# Autodesk Inventor assembly: 810003-XX
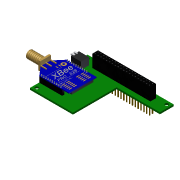
[picture p0: Inventor's stored thumbnail of the model, 180x180]
Saved by Autodesk Inventor 2015 (Build 190159000, 159)
## iProperties
Created: 2014-08-12
Part Number: 810003-XX
Document SubType Name: Assembly
Designer: david
Author: david
## Documents named in this file (6)
- C:\SharedDrive\Dropbox\FAST Robotics\Products\810003_Radio Shield\MECH\810003_Radio Shield\810003A\810003-XX.iam
- C:\SharedDrive\Dropbox\FAST Robotics\Products\810003_Radio Shield\MECH\818001_Radio Shield Bare PCB\818001A\818001A_Radio Shield Bare PCB.ipt
- C:\SharedDrive\Dropbox\FAST Robotics\Library\784005_HEADER Female Socket 10pos 2mm Thru-Hole\784005_HEADER Female Socket 10pos 2mm Thru-Hole.ipt
- C:\SharedDrive\Dropbox\FAST Robotics\Library\616001_DIP Switch Side 2Pos\MECH\616001_DIP Switch Side 2Pos.ipt
- C:\SharedDrive\Dropbox\FAST Robotics\Library\363002_XBee XBP24BZ7SIT\MECH\Imported Components\User Library-XBP24BZ7SIT-004-radio\Assembly2.iam
- C:\SharedDrive\Dropbox\FAST Robotics\Library\784009_PC104 Connector\784009_PC104 Connector.ipt
## Components (6 placed, 5 different names)
1. 818001A_Radio Shield Bare PCB:1 — Flush:1, Flush:2, Flush:3, Mate:3, Mate:4, Flush:14, Flush:15, Flush:16, Flush:17, Mate:9, Flush:18, Mate:10
2. 784005_HEADER Female Socket 10pos 2mm Thru-Hole:1 — Flush:10, Mate:3, Mate:5, Mate:6, Flush:13, Flush:14, Flush:15, Mate:8
3. 784005_HEADER Female Socket 10pos 2mm Thru-Hole:2 — Flush:10, Flush:13, Mate:7
4. 616001_DIP Switch Side 2Pos:1 — Mate:4, Flush:16, Flush:17
5. Assembly2:1 [sub-assembly] — Mate:5, Mate:6, Mate:7, Mate:8
6. 784009_PC104 Connector:1 — Mate:9, Flush:18, Mate:10
## Relationships (18: Flush 10, Mate 8)
- Flush:1: 818001A_Radio Shield Bare PCB:1
- Flush:2: 818001A_Radio Shield Bare PCB:1
- Flush:3: 818001A_Radio Shield Bare PCB:1
- Flush:10: 784005_HEADER Female Socket 10pos 2mm Thru-Hole:1 ↔ 784005_HEADER Female Socket 10pos 2mm Thru-Hole:2
- Mate:3: 818001A_Radio Shield Bare PCB:1 ↔ 784005_HEADER Female Socket 10pos 2mm Thru-Hole:1
- Mate:4: 818001A_Radio Shield Bare PCB:1 ↔ 616001_DIP Switch Side 2Pos:1
- Mate:5: 784005_HEADER Female Socket 10pos 2mm Thru-Hole:1 ↔ Assembly2:1
- Mate:6: 784005_HEADER Female Socket 10pos 2mm Thru-Hole:1 ↔ Assembly2:1
- Flush:13: 784005_HEADER Female Socket 10pos 2mm Thru-Hole:1 ↔ 784005_HEADER Female Socket 10pos 2mm Thru-Hole:2
- Flush:14: 818001A_Radio Shield Bare PCB:1 ↔ 784005_HEADER Female Socket 10pos 2mm Thru-Hole:1
- Mate:7: 784005_HEADER Female Socket 10pos 2mm Thru-Hole:2 ↔ Assembly2:1
- Flush:15 (8.128 mm): 818001A_Radio Shield Bare PCB:1 ↔ 784005_HEADER Female Socket 10pos 2mm Thru-Hole:1
- Mate:8: 784005_HEADER Female Socket 10pos 2mm Thru-Hole:1 ↔ Assembly2:1
- Flush:16: 818001A_Radio Shield Bare PCB:1 ↔ 616001_DIP Switch Side 2Pos:1
- Flush:17 (-7.62 mm): 818001A_Radio Shield Bare PCB:1 ↔ 616001_DIP Switch Side 2Pos:1
- Mate:9: 818001A_Radio Shield Bare PCB:1 ↔ 784009_PC104 Connector:1
- Flush:18 (4.318 mm): 818001A_Radio Shield Bare PCB:1 ↔ 784009_PC104 Connector:1
- Mate:10 (-13.716 mm): 818001A_Radio Shield Bare PCB:1 ↔ 784009_PC104 Connector:1
